# Autodesk Inventor assembly: draft assembly
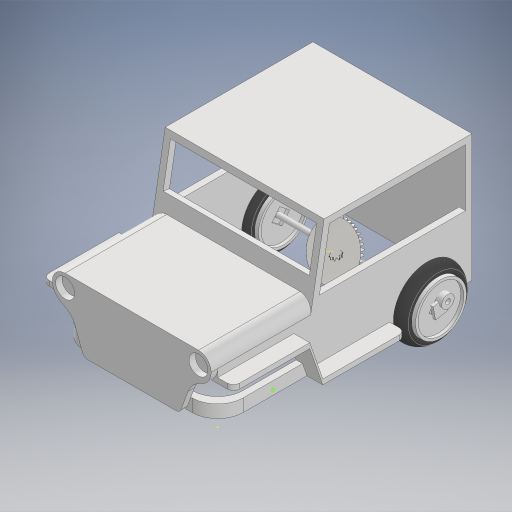
[picture p0: Inventor's stored thumbnail of the model, 512x512]
Saved by Autodesk Inventor 2024 (Build 280153000, 153)
## iProperties
Created: 2024-04-10
Part Number: draft assembly
Document SubType Name: Assembly
Designer: Alex
Author: Alex
## Documents named in this file (7)
- C:\Shared\alex-bartella-schoolwork\4z03\final\draft assembly.iam
- C:\Shared\alex-bartella-schoolwork\4z03\final\tire.ipt
- C:\Shared\alex-bartella-schoolwork\4z03\final\wheel.ipt
- C:\Shared\alex-bartella-schoolwork\4z03\final\shell.ipt
- C:\Shared\alex-bartella-schoolwork\4z03\final\draft assembly\Design Accelerator\Bevel Gears1.iam
- C:\Shared\alex-bartella-schoolwork\4z03\final\draft assembly\Design Accelerator\Bevel Gears4.iam
- C:\Shared\alex-bartella-schoolwork\4z03\final\rear axle.ipt
## Components (8 placed, 5 different names)
1. tire:1 — Mate:1, Mate:2
2. wheel:1 — Mate:1, Mate:2, Flush:3, Mate:11, Mate:13, Mate:14
3. shell:1 — Flush:2, Flush:3, Mate:11, Flush:4
4. tire:2
5. wheel:2 — Flush:2, Mate:12, Mate:13, Flush:4
6. Bevel Gears:1 [sub-assembly]
7. Bevel Gears:2 [sub-assembly] — Mate:12
8. rear axle:1 — Mate:14
## Relationships (11: Mate 8, Flush 3)
- Mate:1: tire:1 ↔ wheel:1
- Mate:2: tire:1 ↔ wheel:1
- [Mate]: tire:2 ↔ wheel:2
- [Mate]: tire:2 ↔ wheel:2
- Flush:2: shell:1 ↔ wheel:2
- Flush:3: wheel:1 ↔ shell:1
- Mate:11: wheel:1 ↔ shell:1
- Mate:12: wheel:2 ↔ Bevel Gears:2
- Mate:13: wheel:1 ↔ wheel:2
- Flush:4: shell:1 ↔ wheel:2
- Mate:14: wheel:1 ↔ rear axle:1
## Named parameters: d2_d0 = 0 mm, d3_d1 = 0 mm
